# Autodesk Inventor assembly: アーム アームユニットアセンブリ
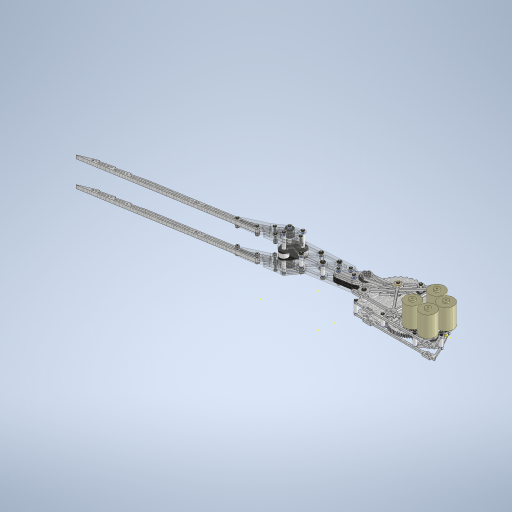
[picture p0: Inventor's stored thumbnail of the model, 512x512]
Saved by Autodesk Inventor 2023 (Build 270158000, 158)
## iProperties
Created: 2020-05-02
Part Number: アーム アームユニットアセンブリ
Document SubType Name: Assembly
Designer: mozar
Mass: 827.78 g
Surface Area: 2311.91 cm^2
Volume: 284.419 cm^3
Density: 2.91042 g/cm^3
Author: mozar
## Documents named in this file (40)
- C:\Users\muzho\Documents\srdc\srdc_2\アーム(世古)\アーム アームユニットアセンブリ.iam
- C:\Users\muzho\Documents\srdc\srdc_2\アーム(世古)\アーム 右フレーム.ipt
- C:\Users\muzho\Documents\srdc\srdc_2\アーム(世古)\アーム 真ん中フレーム.ipt
- C:\Users\muzho\Documents\srdc\srdc_2\アーム(世古)\既製品\アーム　初段焼結ギア　80-10　.ipt
- C:\Users\muzho\Documents\srdc\srdc_2\アーム(世古)\既製品\ベアリング　内径4外径9.ipt
- C:\Users\muzho\Documents\srdc\srdc_2\アーム(世古)\既製品\ベアリング　内径6外径15.ipt
- C:\Users\muzho\Documents\srdc\srdc_2\アーム(世古)\既製品\ドライメットブッシュ 内径6フランジ付き.ipt
- C:\Users\muzho\Documents\srdc\srdc_2\アーム(世古)\既製品\マブチモーター　RS-380PH.ipt
- C:\Users\muzho\Documents\srdc\srdc_2\アーム(世古)\既製品\ピニオン　m0.5　10t.ipt
- C:\Users\muzho\Documents\srdc\srdc_2\アーム(世古)\アーム 最終段ギア36兼駆動節.ipt
- C:\Users\muzho\Documents\srdc\srdc_2\アーム(世古)\アーム 2段目ギアアセンブリ 8 64.ipt.iam
- C:\Users\muzho\Documents\srdc\srdc_2\アーム(世古)\既製品\スペーサーm3-16　簡易筒型.ipt
- C:\Users\muzho\Documents\srdc\srdc_2\アーム(世古)\アーム ツインロッドアーム先端アセンブリ.iam
- C:\Users\muzho\Documents\srdc\srdc_2\アーム(世古)\アーム モーターマウントフレーム.ipt
- C:\Users\muzho\Documents\srdc\srdc_2\アーム(世古)\アーム 左フレーム.ipt
- C:\Users\muzho\Documents\srdc\srdc_2\アーム(世古)\既製品\スペーサーm4-35　簡易筒型.ipt
- C:\Users\muzho\Documents\srdc\srdc_2\アーム(世古)\既製品\チタンワッシャー　4.2-10-1.ipt
- C:\Users\muzho\Documents\srdc\srdc_2\アーム(世古)\既製品\平行ピン　φ4　長さ25.ipt
- C:\Users\muzho\Documents\srdc\srdc_2\アーム(世古)\既製品\平行ピン　φ6　長さ30.ipt
- C:\Users\muzho\Documents\srdc\srdc_2\アーム(世古)\既製品\平行ピン　φ6　長さ25.ipt
- C:\Users\muzho\Documents\srdc\srdc_2\アーム(世古)\既製品\ねじ\SB　6mmなべネジ.ipt
- C:\Users\muzho\Documents\srdc\srdc_2\アーム(世古)\既製品\ねじ\SB　6mm皿ネジ.ipt
- C:\Users\muzho\Documents\srdc\srdc_2\アーム(世古)\アーム 中間節 中詰め.ipt
- C:\Users\muzho\Documents\srdc\srdc_2\アーム(世古)\既製品\ねじ\SB　M4 8mm なべネジ.ipt
- C:\Users\muzho\Documents\srdc\srdc_2\アーム(世古)\既製品\ねじ\SB　8mmなべネジ.ipt
- C:\Users\muzho\Documents\srdc\srdc_2\アーム(世古)\既製品\ねじ\M2.6 ボルト 10mm.ipt
- C:\Users\muzho\Documents\srdc\srdc_2\アーム(世古)\既製品\ねじ\SB　10mmなべネジ.ipt
- C:\Users\muzho\Documents\srdc\srdc_2\アーム(世古)\アーム 駆動フリー節.ipt
- C:\Users\muzho\Documents\srdc\srdc_2\アーム(世古)\アーム 中間節(ミラー).ipt
- C:\Users\muzho\Documents\srdc\srdc_2\アーム(世古)\アーム 揺動節.ipt
- C:\Users\muzho\Documents\srdc\srdc_2\アーム(世古)\アーム 中間節.ipt
- C:\Users\muzho\Documents\srdc\srdc_2\アーム(世古)\アーム 小さいカム押さえるやつ.ipt
- C:\Users\muzho\Documents\srdc\srdc_2\アーム(世古)\アーム 小さいカム.ipt
- C:\Users\muzho\Documents\srdc\srdc_2\アーム(世古)\既製品\ドライメットブッシュ 内径8フランジ付き 2mm.ipt
- C:\Users\muzho\Documents\srdc\srdc_2\アーム(世古)\既製品\ドライメット　内径14 フランジ付き6mm.ipt
- C:\Users\muzho\Documents\srdc\srdc_2\アーム(世古)\既製品\ねじ\SB　25mmなべネジ.ipt
- C:\Users\muzho\Documents\srdc\srdc_2\アーム(世古)\既製品\ねじ\ナイロンナットm3.ipt
- C:\Users\muzho\Documents\srdc\srdc_2\アーム(世古)\既製品\スペーサーm3-14　本物　簡易筒型.ipt
- C:\Users\muzho\Documents\srdc\srdc_2\アーム(世古)\既製品\スペーサーm3-5　簡易筒型.ipt
- アーム 2段目ギアアセンブリ 8 64.ipt
## Components (96 placed, 38 different names)
1. アーム 右フレーム:1 — 挿入:4, 挿入:5, 挿入:70, 挿入:87, 挿入:88, 挿入:89, 挿入:90, 挿入:91, 挿入:93, 挿入:112, 挿入:113, 挿入:132, 挿入:155, 挿入:156
2. アーム 真ん中フレーム:1 — 挿入:3, 挿入:6, 挿入:7, 挿入:11, 挿入:12, 挿入:14, メイト:2, メイト:3, メイト:4, メイト:5, メイト:16, 挿入:65, 挿入:66, 挿入:71, 挿入:74, 挿入:75, 挿入:76, 挿入:77, 挿入:78, 挿入:79, 挿入:95, 挿入:96, 挿入:98, 挿入:99, 挿入:120, 挿入:121, 挿入:122, 挿入:123, 挿入:124, 挿入:125, 挿入:126, 挿入:127, 挿入:131, 挿入:133, 挿入:159
3. アーム　初段焼結ギア　80-10　:1 — 挿入:15
4. ベアリング　内径4外径9:1 — 挿入:4, 挿入:84
5. ベアリング　内径4外径9:2 — 挿入:3, 挿入:15
6. ベアリング　内径6外径15:1 — 挿入:18, 挿入:70, 挿入:85
7. ベアリング　内径6外径15:2 — 挿入:16, 挿入:71
8. ドライメットブッシュ 内径6フランジ付き:1 — 挿入:5, メイト:1
9. ドライメットブッシュ 内径6フランジ付き:2 — 挿入:6, 挿入:17, メイト:1, 挿入:86
10. マブチモーター　RS-380PH:1 — 挿入:7, 挿入:22, メイト:4
11. マブチモーター　RS-380PH:2 — 挿入:12, 挿入:20, メイト:3
12. マブチモーター　RS-380PH:3 — 挿入:11, 挿入:19, メイト:2
13. マブチモーター　RS-380PH:4 — 挿入:14, 挿入:21, メイト:5
14. ピニオン　m0.5　10t:1 — 挿入:21
15. ピニオン　m0.5　10t:2 — 挿入:19
16. ピニオン　m0.5　10t:3 — 挿入:20
17. ピニオン　m0.5　10t:4 — 挿入:22
18. アーム 最終段ギア36兼駆動節:1 — 挿入:17, 挿入:138, メイト:46, 挿入:149, 挿入:150, 挿入:151
19. アーム 2段目ギアアセンブリ 8 64.ipt:1 [sub-assembly] — 挿入:16, 挿入:18
20. スペーサーm3-16　簡易筒型:1 — 挿入:64
21. スペーサーm3-16　簡易筒型:2 — 挿入:143, メイト:50
22. スペーサーm3-16　簡易筒型:3 — 挿入:63, メイト:48
23. ドライメットブッシュ 内径6フランジ付き:3 — メイト:16, 挿入:140
24. アーム ツインロッドアーム先端アセンブリ:1 [sub-assembly] — 挿入:63, 挿入:64, メイト:37, 挿入:114, 挿入:115, 挿入:116, 挿入:117, 挿入:118, 挿入:119, メイト:49, 挿入:143
25. アーム モーターマウントフレーム:1 — 挿入:65, 挿入:66, 挿入:109, 挿入:128, 挿入:129, 挿入:130
26. アーム 左フレーム:1 — 挿入:68, 挿入:97, 挿入:110, 挿入:111, 挿入:157, 挿入:158
27. ドライメットブッシュ 内径6フランジ付き:4 — 挿入:68
28. スペーサーm4-35　簡易筒型:1 — 挿入:155, 挿入:158
29. スペーサーm4-35　簡易筒型:2 — 挿入:156, 挿入:157, 正接:1
30. スペーサーm3-16　簡易筒型:1 — 挿入:131
31. スペーサーm3-16　簡易筒型:3 — 挿入:79
32. スペーサーm3-16　簡易筒型:6 — 挿入:75
33. スペーサーm3-16　簡易筒型:7 — 挿入:76
34. スペーサーm3-16　簡易筒型:8 — 挿入:77
35. スペーサーm3-16　簡易筒型:9 — 挿入:78
36. スペーサーm3-16　簡易筒型:10 — 挿入:74
37. チタンワッシャー　4.2-10-1:1 — 挿入:161, 挿入:162
38. 平行ピン　φ4　長さ25:1 — 挿入:84
39. 平行ピン　φ6　長さ30:1 — 挿入:85
40. 平行ピン　φ6　長さ25:1 — 挿入:86
41. SB　6mmなべネジ:1 — 挿入:133
42. SB　6mmなべネジ:2 — 挿入:93
43. SB　6mmなべネジ:3 — 挿入:96
44. SB　6mmなべネジ:4 — 挿入:97
45. SB　6mmなべネジ:5 — 挿入:95
46. SB　6mmなべネジ:7 — 挿入:98
47. SB　6mmなべネジ:8 — 挿入:91
48. SB　6mmなべネジ:9 — 挿入:90
49. SB　6mmなべネジ:10 — 挿入:132
50. SB　6mmなべネジ:11 — 挿入:89
51. SB　6mmなべネジ:12 — 挿入:88
52. SB　6mmなべネジ:13 — 挿入:87
53. SB　6mm皿ネジ:1 — 挿入:99
54. アーム 中間節 中詰め:1 — 挿入:104, 挿入:105, メイト:37, メイト:49
55. アーム 中間節 中詰め:2 — 挿入:104, 挿入:105, 挿入:142
56. SB　6mm皿ネジ:2 — 挿入:148
57. SB　6mm皿ネジ:3 — 挿入:147
58. SB　6mmなべネジ:14 — 挿入:109
59. SB　M4 8mm なべネジ:1 — 挿入:111
60. SB　M4 8mm なべネジ:2 — 挿入:113
61. SB　M4 8mm なべネジ:3 — 挿入:112
62. SB　M4 8mm なべネジ:4 — 挿入:110
63. SB　8mmなべネジ:1 — 挿入:115
64. SB　8mmなべネジ:2 — 挿入:114
65. SB　8mmなべネジ:3 — 挿入:116
66. SB　8mmなべネジ:4 — 挿入:118
67. SB　8mmなべネジ:5 — 挿入:117
68. SB　8mmなべネジ:6 — 挿入:119
69. M2.6 ボルト 10mm:1 — 挿入:122
70. M2.6 ボルト 10mm:2 — 挿入:124
71. M2.6 ボルト 10mm:3 — 挿入:123
72. M2.6 ボルト 10mm:4 — 挿入:126
73. M2.6 ボルト 10mm:5 — 挿入:127
74. M2.6 ボルト 10mm:6 — 挿入:125
75. M2.6 ボルト 10mm:7 — 挿入:120
76. M2.6 ボルト 10mm:8 — 挿入:121
77. SB　10mmなべネジ:1 — 挿入:130
78. SB　10mmなべネジ:2 — 挿入:129
79. SB　10mmなべネジ:3 — 挿入:128
80. アーム 駆動フリー節:1 — 挿入:144, メイト:51, 挿入:152, 挿入:153, 挿入:154, メイト:52, メイト:53, メイト:54, 挿入:160
81. アーム 中間節(ミラー):1 — 挿入:136, メイト:45, 挿入:137, メイト:48, 挿入:147, 挿入:148
82. アーム 揺動節:1 — 挿入:134, 挿入:140
83. アーム 中間節:1 — 挿入:135, 挿入:136, メイト:45, 挿入:142, メイト:50, 正接:1
84. アーム 小さいカム押さえるやつ:1 — 挿入:138, メイト:46, 挿入:139, メイト:47
85. アーム 小さいカム:1 — 挿入:139, メイト:47, 挿入:141, 挿入:144, メイト:51
86. ドライメットブッシュ 内径8フランジ付き 2mm:1 — 挿入:134, 挿入:135
87. ドライメット　内径14 フランジ付き6mm:1 — 挿入:137, 挿入:141
88. SB　25mmなべネジ:1 — 挿入:149
89. SB　25mmなべネジ:2 — 挿入:150
90. SB　25mmなべネジ:3 — 挿入:151
91. ナイロンナットm3:1 — 挿入:152, メイト:52
92. ナイロンナットm3:2 — 挿入:153, メイト:54
93. ナイロンナットm3:3 — 挿入:154, メイト:53
94. スペーサーm3-14　本物　簡易筒型:1 — 挿入:159
95. スペーサーm3-5　簡易筒型:1 — 挿入:160, 挿入:161
96. SB　10mmなべネジ:4 — 挿入:162
## Relationships (115: Insert 97, Mate 17, Tangent 1)
- 挿入:3 [Insert]: アーム 真ん中フレーム:1 ↔ ベアリング　内径4外径9:2
- 挿入:4 [Insert]: アーム 右フレーム:1 ↔ ベアリング　内径4外径9:1
- 挿入:5 [Insert]: アーム 右フレーム:1 ↔ ドライメットブッシュ 内径6フランジ付き:1
- 挿入:6 [Insert]: アーム 真ん中フレーム:1 ↔ ドライメットブッシュ 内径6フランジ付き:2
- 挿入:7 [Insert] (4 mm): アーム 真ん中フレーム:1 ↔ マブチモーター　RS-380PH:1
- 挿入:11 [Insert] (4 mm): アーム 真ん中フレーム:1 ↔ マブチモーター　RS-380PH:3
- 挿入:12 [Insert] (4 mm): アーム 真ん中フレーム:1 ↔ マブチモーター　RS-380PH:2
- 挿入:14 [Insert] (4 mm): アーム 真ん中フレーム:1 ↔ マブチモーター　RS-380PH:4
- 挿入:15 [Insert] (6 mm): アーム　初段焼結ギア　80-10　:1 ↔ ベアリング　内径4外径9:2
- 挿入:16 [Insert] (1.6 mm): ベアリング　内径6外径15:2 ↔ アーム 2段目ギアアセンブリ 8 64.ipt:1
- 挿入:17 [Insert] (0.6 mm): ドライメットブッシュ 内径6フランジ付き:2 ↔ アーム 最終段ギア36兼駆動節:1
- 挿入:18 [Insert] (1 mm): ベアリング　内径6外径15:1 ↔ アーム 2段目ギアアセンブリ 8 64.ipt:1
- メイト:1 [Mate]: ドライメットブッシュ 内径6フランジ付き:1 ↔ ドライメットブッシュ 内径6フランジ付き:2
- 挿入:19 [Insert]: マブチモーター　RS-380PH:3 ↔ ピニオン　m0.5　10t:2
- 挿入:20 [Insert]: マブチモーター　RS-380PH:2 ↔ ピニオン　m0.5　10t:3
- 挿入:21 [Insert]: マブチモーター　RS-380PH:4 ↔ ピニオン　m0.5　10t:1
- 挿入:22 [Insert]: マブチモーター　RS-380PH:1 ↔ ピニオン　m0.5　10t:4
- メイト:2 [Mate]: アーム 真ん中フレーム:1 ↔ マブチモーター　RS-380PH:3
- メイト:3 [Mate]: アーム 真ん中フレーム:1 ↔ マブチモーター　RS-380PH:2
- メイト:4 [Mate]: アーム 真ん中フレーム:1 ↔ マブチモーター　RS-380PH:1
- メイト:5 [Mate]: アーム 真ん中フレーム:1 ↔ マブチモーター　RS-380PH:4
- メイト:16 [Mate]: アーム 真ん中フレーム:1 ↔ ドライメットブッシュ 内径6フランジ付き:3
- 挿入:63 [Insert]: スペーサーm3-16　簡易筒型:3 ↔ アーム ツインロッドアーム先端アセンブリ:1
- 挿入:64 [Insert]: スペーサーm3-16　簡易筒型:1 ↔ アーム ツインロッドアーム先端アセンブリ:1
- 挿入:65 [Insert]: アーム 真ん中フレーム:1 ↔ アーム モーターマウントフレーム:1
- 挿入:66 [Insert]: アーム 真ん中フレーム:1 ↔ アーム モーターマウントフレーム:1
- 挿入:68 [Insert]: アーム 左フレーム:1 ↔ ドライメットブッシュ 内径6フランジ付き:4
- 挿入:70 [Insert]: アーム 右フレーム:1 ↔ ベアリング　内径6外径15:1
- 挿入:71 [Insert]: アーム 真ん中フレーム:1 ↔ ベアリング　内径6外径15:2
- 挿入:74 [Insert]: アーム 真ん中フレーム:1 ↔ スペーサーm3-16　簡易筒型:10
- 挿入:75 [Insert]: アーム 真ん中フレーム:1 ↔ スペーサーm3-16　簡易筒型:6
- 挿入:76 [Insert]: アーム 真ん中フレーム:1 ↔ スペーサーm3-16　簡易筒型:7
- 挿入:77 [Insert]: アーム 真ん中フレーム:1 ↔ スペーサーm3-16　簡易筒型:8
- 挿入:78 [Insert]: アーム 真ん中フレーム:1 ↔ スペーサーm3-16　簡易筒型:9
- 挿入:79 [Insert]: アーム 真ん中フレーム:1 ↔ スペーサーm3-16　簡易筒型:3
- 挿入:84 [Insert]: ベアリング　内径4外径9:1 ↔ 平行ピン　φ4　長さ25:1
- 挿入:85 [Insert]: ベアリング　内径6外径15:1 ↔ 平行ピン　φ6　長さ30:1
- 挿入:86 [Insert]: ドライメットブッシュ 内径6フランジ付き:2 ↔ 平行ピン　φ6　長さ25:1
- 挿入:87 [Insert]: アーム 右フレーム:1 ↔ SB　6mmなべネジ:13
- 挿入:88 [Insert]: アーム 右フレーム:1 ↔ SB　6mmなべネジ:12
- 挿入:89 [Insert]: アーム 右フレーム:1 ↔ SB　6mmなべネジ:11
- 挿入:90 [Insert]: アーム 右フレーム:1 ↔ SB　6mmなべネジ:9
- 挿入:91 [Insert]: アーム 右フレーム:1 ↔ SB　6mmなべネジ:8
- 挿入:93 [Insert]: アーム 右フレーム:1 ↔ SB　6mmなべネジ:2
- 挿入:95 [Insert]: アーム 真ん中フレーム:1 ↔ SB　6mmなべネジ:5
- 挿入:96 [Insert]: アーム 真ん中フレーム:1 ↔ SB　6mmなべネジ:3
- 挿入:97 [Insert]: アーム 左フレーム:1 ↔ SB　6mmなべネジ:4
- 挿入:98 [Insert]: アーム 真ん中フレーム:1 ↔ SB　6mmなべネジ:7
- 挿入:99 [Insert]: アーム 真ん中フレーム:1 ↔ SB　6mm皿ネジ:1
- 挿入:104 [Insert]: アーム 中間節 中詰め:1 ↔ アーム 中間節 中詰め:2
- 挿入:105 [Insert]: アーム 中間節 中詰め:1 ↔ アーム 中間節 中詰め:2
- メイト:37 [Mate]: アーム ツインロッドアーム先端アセンブリ:1 ↔ アーム 中間節 中詰め:1
- 挿入:109 [Insert]: アーム モーターマウントフレーム:1 ↔ SB　6mmなべネジ:14
- 挿入:110 [Insert]: アーム 左フレーム:1 ↔ SB　M4 8mm なべネジ:4
- 挿入:111 [Insert]: アーム 左フレーム:1 ↔ SB　M4 8mm なべネジ:1
- 挿入:112 [Insert]: アーム 右フレーム:1 ↔ SB　M4 8mm なべネジ:3
- 挿入:113 [Insert]: アーム 右フレーム:1 ↔ SB　M4 8mm なべネジ:2
- 挿入:114 [Insert]: アーム ツインロッドアーム先端アセンブリ:1 ↔ SB　8mmなべネジ:2
- 挿入:115 [Insert]: アーム ツインロッドアーム先端アセンブリ:1 ↔ SB　8mmなべネジ:1
- 挿入:116 [Insert]: アーム ツインロッドアーム先端アセンブリ:1 ↔ SB　8mmなべネジ:3
- 挿入:117 [Insert]: アーム ツインロッドアーム先端アセンブリ:1 ↔ SB　8mmなべネジ:5
- 挿入:118 [Insert]: アーム ツインロッドアーム先端アセンブリ:1 ↔ SB　8mmなべネジ:4
- 挿入:119 [Insert]: アーム ツインロッドアーム先端アセンブリ:1 ↔ SB　8mmなべネジ:6
- 挿入:120 [Insert]: アーム 真ん中フレーム:1 ↔ M2.6 ボルト 10mm:7
- 挿入:121 [Insert]: アーム 真ん中フレーム:1 ↔ M2.6 ボルト 10mm:8
- 挿入:122 [Insert]: アーム 真ん中フレーム:1 ↔ M2.6 ボルト 10mm:1
- 挿入:123 [Insert]: アーム 真ん中フレーム:1 ↔ M2.6 ボルト 10mm:3
- 挿入:124 [Insert]: アーム 真ん中フレーム:1 ↔ M2.6 ボルト 10mm:2
- 挿入:125 [Insert]: アーム 真ん中フレーム:1 ↔ M2.6 ボルト 10mm:6
- 挿入:126 [Insert]: アーム 真ん中フレーム:1 ↔ M2.6 ボルト 10mm:4
- 挿入:127 [Insert]: アーム 真ん中フレーム:1 ↔ M2.6 ボルト 10mm:5
- 挿入:128 [Insert]: アーム モーターマウントフレーム:1 ↔ SB　10mmなべネジ:3
- 挿入:129 [Insert]: アーム モーターマウントフレーム:1 ↔ SB　10mmなべネジ:2
- 挿入:130 [Insert]: アーム モーターマウントフレーム:1 ↔ SB　10mmなべネジ:1
- 挿入:131 [Insert]: アーム 真ん中フレーム:1 ↔ スペーサーm3-16　簡易筒型:1
- 挿入:132 [Insert]: アーム 右フレーム:1 ↔ SB　6mmなべネジ:10
- 挿入:133 [Insert]: アーム 真ん中フレーム:1 ↔ SB　6mmなべネジ:1
- 挿入:134 [Insert]: アーム 揺動節:1 ↔ ドライメットブッシュ 内径8フランジ付き 2mm:1
- 挿入:135 [Insert] (0.25 mm): アーム 中間節:1 ↔ ドライメットブッシュ 内径8フランジ付き 2mm:1
- 挿入:136 [Insert]: アーム 中間節(ミラー):1 ↔ アーム 中間節:1
- メイト:45 [Mate]: アーム 中間節(ミラー):1 ↔ アーム 中間節:1
- 挿入:137 [Insert]: アーム 中間節(ミラー):1 ↔ ドライメット　内径14 フランジ付き6mm:1
- 挿入:138 [Insert]: アーム 最終段ギア36兼駆動節:1 ↔ アーム 小さいカム押さえるやつ:1
- メイト:46 [Mate]: アーム 最終段ギア36兼駆動節:1 ↔ アーム 小さいカム押さえるやつ:1
- 挿入:139 [Insert]: アーム 小さいカム押さえるやつ:1 ↔ アーム 小さいカム:1
- メイト:47 [Mate]: アーム 小さいカム押さえるやつ:1 ↔ アーム 小さいカム:1
- 挿入:140 [Insert]: ドライメットブッシュ 内径6フランジ付き:3 ↔ アーム 揺動節:1
- 挿入:141 [Insert] (0.5 mm): アーム 小さいカム:1 ↔ ドライメット　内径14 フランジ付き6mm:1
- 挿入:142 [Insert]: アーム 中間節 中詰め:2 ↔ アーム 中間節:1
- メイト:48 [Mate]: スペーサーm3-16　簡易筒型:3 ↔ アーム 中間節(ミラー):1
- メイト:49 [Mate]: アーム ツインロッドアーム先端アセンブリ:1 ↔ アーム 中間節 中詰め:1
- 挿入:143 [Insert]: スペーサーm3-16　簡易筒型:2 ↔ アーム ツインロッドアーム先端アセンブリ:1
- メイト:50 [Mate]: スペーサーm3-16　簡易筒型:2 ↔ アーム 中間節:1
- 挿入:144 [Insert]: アーム 駆動フリー節:1 ↔ アーム 小さいカム:1
- メイト:51 [Mate]: アーム 駆動フリー節:1 ↔ アーム 小さいカム:1
- 挿入:147 [Insert]: SB　6mm皿ネジ:3 ↔ アーム 中間節(ミラー):1
- 挿入:148 [Insert]: SB　6mm皿ネジ:2 ↔ アーム 中間節(ミラー):1
- 挿入:149 [Insert]: アーム 最終段ギア36兼駆動節:1 ↔ SB　25mmなべネジ:1
- 挿入:150 [Insert]: アーム 最終段ギア36兼駆動節:1 ↔ SB　25mmなべネジ:2
- 挿入:151 [Insert]: アーム 最終段ギア36兼駆動節:1 ↔ SB　25mmなべネジ:3
- 挿入:152 [Insert]: アーム 駆動フリー節:1 ↔ ナイロンナットm3:1
- 挿入:153 [Insert]: アーム 駆動フリー節:1 ↔ ナイロンナットm3:2
- 挿入:154 [Insert]: アーム 駆動フリー節:1 ↔ ナイロンナットm3:3
- メイト:52 [Mate]: アーム 駆動フリー節:1 ↔ ナイロンナットm3:1
- メイト:53 [Mate]: アーム 駆動フリー節:1 ↔ ナイロンナットm3:3
- メイト:54 [Mate]: アーム 駆動フリー節:1 ↔ ナイロンナットm3:2
- 挿入:155 [Insert]: アーム 右フレーム:1 ↔ スペーサーm4-35　簡易筒型:1
- 挿入:156 [Insert]: アーム 右フレーム:1 ↔ スペーサーm4-35　簡易筒型:2
- 挿入:157 [Insert]: アーム 左フレーム:1 ↔ スペーサーm4-35　簡易筒型:2
- 挿入:158 [Insert]: アーム 左フレーム:1 ↔ スペーサーm4-35　簡易筒型:1
- 挿入:159 [Insert]: アーム 真ん中フレーム:1 ↔ スペーサーm3-14　本物　簡易筒型:1
- 挿入:160 [Insert]: アーム 駆動フリー節:1 ↔ スペーサーm3-5　簡易筒型:1
- 挿入:161 [Insert]: チタンワッシャー　4.2-10-1:1 ↔ スペーサーm3-5　簡易筒型:1
- 挿入:162 [Insert]: チタンワッシャー　4.2-10-1:1 ↔ SB　10mmなべネジ:4
- 正接:1 [Tangent]: スペーサーm4-35　簡易筒型:2 ↔ アーム 中間節:1
